# Autodesk Inventor assembly: extension arm assembly jack
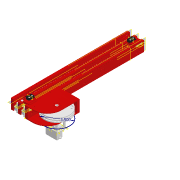
[picture p0: Inventor's stored thumbnail of the model, 180x180]
Saved by Autodesk Inventor 2020 (Build 240168000, 168)
## iProperties
Created: 2020-01-01
Part Number: extension arm assembly jack
Document SubType Name: Assembly
Designer: ball
Author: ball
## Documents named in this file (8)
- C:\FTC\FTC8863CAD\2019 Robot\Delivery\extension arm\extension arm assembly jack.iam
- C:\FTC\FTC8863CAD\2019 Robot\Delivery\extension arm\extension arm top.iam
- C:\FTC\FTC8863CAD\2019 Robot\Delivery\extension arm\extension arm middle.iam
- C:\FTC\FTC8863CAD\2019 Robot\Delivery\extension arm\extension arm bottom.iam
- C:\FTC\FTC8863CAD\2019 Robot\Delivery\extension arm\Servo mount + servo.iam
- C:\FTC\FTC8863CAD\2019 Robot\Delivery\Limit switch top + mount left.iam
- C:\FTC\FTC8863CAD\2019 Robot\Delivery\Lift Right\Limit switch top + mount right.iam
- C:\FTC\FTC8863CAD\2019 Robot\Delivery\extension arm\Limit switch trigger spacer extension arm.ipt
## Components (7 placed, 7 different names)
1. extension arm top:1 [sub-assembly] — Mate:1, Mate:3, Mate:4, Mate:5, Mate:9, Mate:10, Mate:11, Mate:12, Mate:17, Mate:18, Mate:19
2. extension arm middle:1 [sub-assembly] — Mate:1, Mate:2, Mate:3, Mate:4, Mate:5, Mate:6, Mate:7, Mate:8, Mate:23, Mate:24, Mate:25
3. extension arm bottom:1 [sub-assembly] — Mate:2, Mate:6, Mate:7, Mate:8
4. Servo mount + servo:1 [sub-assembly] — Mate:9, Mate:10, Mate:11, Mate:12, Mate:20, Mate:21, Mate:22
5. Limit switch top + mount left:1 [sub-assembly] — Mate:17, Mate:18, Mate:19
6. Limit switch top + mount right:1 [sub-assembly] — Mate:20, Mate:21, Mate:22
7. Limit switch trigger spacer extension arm:1 — Mate:23, Mate:24, Mate:25
## Relationships (21: Mate 21)
- Mate:1: extension arm top:1 ↔ extension arm middle:1
- Mate:2: extension arm middle:1 ↔ extension arm bottom:1
- Mate:3: extension arm top:1 ↔ extension arm middle:1
- Mate:4: extension arm top:1 ↔ extension arm middle:1
- Mate:5: extension arm top:1 ↔ extension arm middle:1
- Mate:6: extension arm middle:1 ↔ extension arm bottom:1
- Mate:7: extension arm middle:1 ↔ extension arm bottom:1
- Mate:8: extension arm middle:1 ↔ extension arm bottom:1
- Mate:9: extension arm top:1 ↔ Servo mount + servo:1
- Mate:10: extension arm top:1 ↔ Servo mount + servo:1
- Mate:11: extension arm top:1 ↔ Servo mount + servo:1
- Mate:12: extension arm top:1 ↔ Servo mount + servo:1
- Mate:17: extension arm top:1 ↔ Limit switch top + mount left:1
- Mate:18: extension arm top:1 ↔ Limit switch top + mount left:1
- Mate:19: extension arm top:1 ↔ Limit switch top + mount left:1
- Mate:20: Servo mount + servo:1 ↔ Limit switch top + mount right:1
- Mate:21: Servo mount + servo:1 ↔ Limit switch top + mount right:1
- Mate:22: Servo mount + servo:1 ↔ Limit switch top + mount right:1
- Mate:23: extension arm middle:1 ↔ Limit switch trigger spacer extension arm:1
- Mate:24: extension arm middle:1 ↔ Limit switch trigger spacer extension arm:1
- Mate:25: extension arm middle:1 ↔ Limit switch trigger spacer extension arm:1
